# Autodesk Inventor assembly: 40TShaft_RearSide
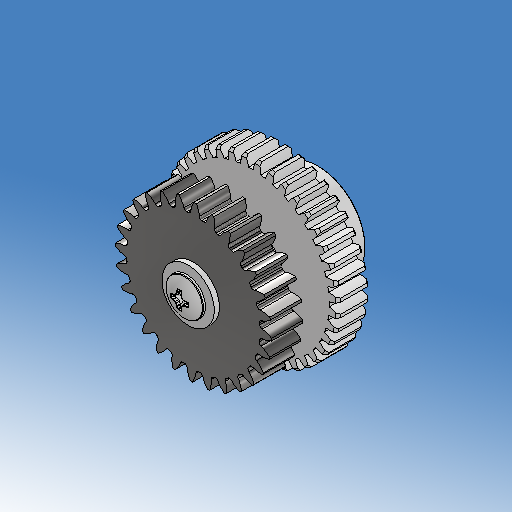
[picture p0: Inventor's stored thumbnail of the model, 512x512]
Saved by Autodesk Inventor 2025 (Build 290162000, 162)
## iProperties
Created: 2024-06-13
Part Number: 40TShaft_RearSide
Document SubType Name: Assembly
Designer: seene
Author: seene
## Documents named in this file (8)
- C:\Users\seene\OneDrive\SBRT\Robocup Rescue\Drive\v1\40TShaft_RearSide.iam
- C:\Users\seene\OneDrive\SBRT\Robocup Rescue\Drive\v1\1.5inRoundHexShaft.ipt
- C:\Users\seene\OneDrive\SBRT\Robocup Rescue\Drive\v1\am-3948-063 500H x 063IN Spacer.ipt
- C:\Users\seene\OneDrive\SBRT\Robocup Rescue\Drive\v1\2879T1_High-Load Oil-Embedded 863 Bronze Thrust Bearing.ipt
- C:\Users\seene\OneDrive\SBRT\Robocup Rescue\Drive\v1\91770A830_Extra-Wide Truss Head Phillips Screws.ipt
- C:\Users\seene\OneDrive\SBRT\Robocup Rescue\Drive\v1\REV-21-1916.ipt
- C:\Users\seene\OneDrive\SBRT\Robocup Rescue\Drive\v1\Gears\am-4710 40T 20DP 500hex 375 FW.ipt
- C:\Users\seene\OneDrive\SBRT\Robocup Rescue\Drive\v1\Spur Gear (28 teeth).ipt
## Components (9 placed, 7 different names)
1. 1.5inRoundHexShaft:1 — Mate:1, Flush:1, Mate:2, Mate:4, Mate:6, Mate:7, Flush:2, Mate:12, Mate:13, Mate:14, Mate:15
2. am-3948-063 500H x 063IN Spacer:1 — Mate:2, Mate:3, Mate:5
3. 2879T1_High-Load Oil-Embedded 863 Bronze Thrust Bearing:1 — Mate:8, Mate:9, Mate:12, Mate:15
4. 91770A830_Extra-Wide Truss Head Phillips Screws:1 — Mate:8, Mate:9
5. REV-21-1916:1 — Mate:1, Flush:1, Mate:3
6. am-4710 40T 20DP 500hex 375 FW:1 — Mate:4, Mate:5
7. Spur Gear (28 teeth):1 — Mate:6, Mate:7, Flush:2
8. 2879T1_High-Load Oil-Embedded 863 Bronze Thrust Bearing:2 — Mate:13, Mate:14
9. 91770A830_Extra-Wide Truss Head Phillips Screws:2
## Relationships (17: Mate 15, Flush 2)
- Mate:1: 1.5inRoundHexShaft:1 ↔ REV-21-1916:1
- Flush:1: 1.5inRoundHexShaft:1 ↔ REV-21-1916:1
- Mate:2: 1.5inRoundHexShaft:1 ↔ am-3948-063 500H x 063IN Spacer:1
- Mate:3: am-3948-063 500H x 063IN Spacer:1 ↔ REV-21-1916:1
- Mate:4: 1.5inRoundHexShaft:1 ↔ am-4710 40T 20DP 500hex 375 FW:1
- Mate:5: am-3948-063 500H x 063IN Spacer:1 ↔ am-4710 40T 20DP 500hex 375 FW:1
- Mate:6: 1.5inRoundHexShaft:1 ↔ Spur Gear (28 teeth):1
- Mate:7: 1.5inRoundHexShaft:1 ↔ Spur Gear (28 teeth):1
- Flush:2: 1.5inRoundHexShaft:1 ↔ Spur Gear (28 teeth):1
- Mate:8: 2879T1_High-Load Oil-Embedded 863 Bronze Thrust Bearing:1 ↔ 91770A830_Extra-Wide Truss Head Phillips Screws:1
- Mate:9: 2879T1_High-Load Oil-Embedded 863 Bronze Thrust Bearing:1 ↔ 91770A830_Extra-Wide Truss Head Phillips Screws:1
- [Mate]: 2879T1_High-Load Oil-Embedded 863 Bronze Thrust Bearing:2 ↔ 91770A830_Extra-Wide Truss Head Phillips Screws:2
- [Mate]: 2879T1_High-Load Oil-Embedded 863 Bronze Thrust Bearing:2 ↔ 91770A830_Extra-Wide Truss Head Phillips Screws:2
- Mate:12: 1.5inRoundHexShaft:1 ↔ 2879T1_High-Load Oil-Embedded 863 Bronze Thrust Bearing:1
- Mate:13: 1.5inRoundHexShaft:1 ↔ 2879T1_High-Load Oil-Embedded 863 Bronze Thrust Bearing:2
- Mate:14: 1.5inRoundHexShaft:1 ↔ 2879T1_High-Load Oil-Embedded 863 Bronze Thrust Bearing:2
- Mate:15: 1.5inRoundHexShaft:1 ↔ 2879T1_High-Load Oil-Embedded 863 Bronze Thrust Bearing:1
## Named parameters: d11_d9 = 0 mm, d12_d10 = 0 mm
